# Autodesk Inventor assembly: Box_Assembly
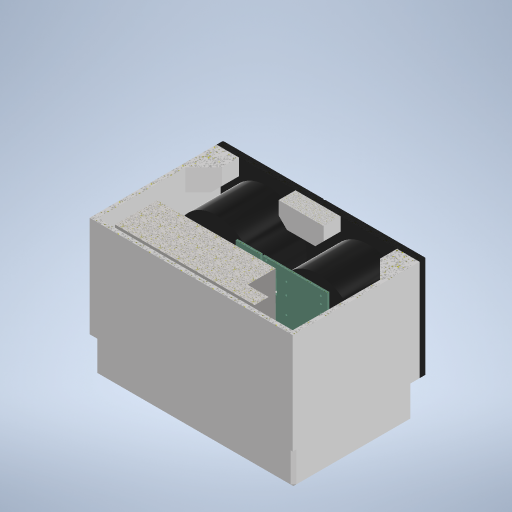
[picture p0: Inventor's stored thumbnail of the model, 512x512]
Saved by Autodesk Inventor 2024 (Build 280153000, 153)
## iProperties
Created: 2026-05-31
Part Number: Box_Assembly
Document SubType Name: Assembly
Designer: maxim
Author: maxim
## Documents named in this file (9)
- D:\maxim\Documents\Nextcloud\Documents\Uni\Semester_10\ES\Morli_Box\Box_Assembly.iam
- D:\maxim\Documents\Nextcloud\Documents\Uni\Semester_10\ES\Morli_Box\Box.ipt
- D:\maxim\Documents\Nextcloud\Documents\Uni\Semester_10\ES\Morli_Box\PSU.ipt
- D:\maxim\Documents\Nextcloud\Documents\Uni\Semester_10\ES\Morli_Box\Kaltstecker.ipt
- D:\maxim\Documents\Nextcloud\Documents\Uni\Semester_10\ES\Morli_Box\Steckdose.ipt
- D:\maxim\Documents\Nextcloud\Documents\Uni\Semester_10\ES\Morli_Box\Steckdosen_Block.ipt
- D:\maxim\Documents\Nextcloud\Documents\Uni\Semester_10\ES\Morli_Box\main_pcb\terrasense_PCB.ipt
- D:\maxim\Documents\Nextcloud\Documents\Uni\Semester_10\ES\Morli_Box\LV_Deckel.ipt
- D:\maxim\Documents\Nextcloud\Documents\Uni\Semester_10\ES\Morli_Box\hv_pcb\high_volt_switch_PCB.ipt
## Components (11 placed, 8 different names)
1. Box:1 — Passend:5, Passend:6, Passend:7, Passend:13, Passend:14, Passend:15, Passend:16, Passend:17, Passend:18, Passend:19, Passend:20, Passend:21, Passend:22, Passend:23, Passend:24, Passend:28, Passend:29, Passend:30, Passend:31, Passend:32, Passend:33, Passend:34, Passend:35, Passend:36, Passend:37, Passend:38, Passend:39
2. PSU:1 — Passend:28, Passend:29, Passend:30
3. Kaltstecker:1 — Passend:5, Passend:6, Passend:7
4. Steckdose:1 — Passend:13, Passend:17, Passend:18, Passend:25, Passend:26
5. Steckdose:2 — Passend:14, Passend:19, Passend:20
6. Steckdose:3 — Passend:15, Passend:21, Passend:22
7. Steckdose:4 — Passend:16, Passend:23, Passend:24, Passend:27
8. Steckdosen_Block:1 — Passend:25, Passend:26, Passend:27
9. terrasense_PCB:1 — Passend:31, Passend:32, Passend:33
10. LV_Deckel:1 — Passend:34, Passend:35, Passend:36
11. high_volt_switch_PCB:1 — Passend:37, Passend:38, Passend:39
## Relationships (30: Mate 30)
- Passend:5 [Mate]: Box:1 ↔ Kaltstecker:1
- Passend:6 [Mate]: Box:1 ↔ Kaltstecker:1
- Passend:7 [Mate]: Box:1 ↔ Kaltstecker:1
- Passend:13 [Mate]: Box:1 ↔ Steckdose:1
- Passend:14 [Mate]: Box:1 ↔ Steckdose:2
- Passend:15 [Mate]: Box:1 ↔ Steckdose:3
- Passend:16 [Mate]: Box:1 ↔ Steckdose:4
- Passend:17 [Mate]: Box:1 ↔ Steckdose:1
- Passend:18 [Mate]: Box:1 ↔ Steckdose:1
- Passend:19 [Mate]: Box:1 ↔ Steckdose:2
- Passend:20 [Mate]: Box:1 ↔ Steckdose:2
- Passend:21 [Mate]: Box:1 ↔ Steckdose:3
- Passend:22 [Mate]: Box:1 ↔ Steckdose:3
- Passend:23 [Mate]: Box:1 ↔ Steckdose:4
- Passend:24 [Mate]: Box:1 ↔ Steckdose:4
- Passend:25 [Mate]: Steckdose:1 ↔ Steckdosen_Block:1
- Passend:26 [Mate]: Steckdose:1 ↔ Steckdosen_Block:1
- Passend:27 [Mate]: Steckdose:4 ↔ Steckdosen_Block:1
- Passend:28 [Mate]: Box:1 ↔ PSU:1
- Passend:29 [Mate]: Box:1 ↔ PSU:1
- Passend:30 [Mate]: Box:1 ↔ PSU:1
- Passend:31 [Mate]: Box:1 ↔ terrasense_PCB:1
- Passend:32 [Mate]: Box:1 ↔ terrasense_PCB:1
- Passend:33 [Mate]: Box:1 ↔ terrasense_PCB:1
- Passend:34 [Mate]: Box:1 ↔ LV_Deckel:1
- Passend:35 [Mate]: Box:1 ↔ LV_Deckel:1
- Passend:36 [Mate]: Box:1 ↔ LV_Deckel:1
- Passend:37 [Mate]: Box:1 ↔ high_volt_switch_PCB:1
- Passend:38 [Mate]: Box:1 ↔ high_volt_switch_PCB:1
- Passend:39 [Mate]: Box:1 ↔ high_volt_switch_PCB:1
